# Autodesk Inventor assembly: (FINAL)rollerAssembly
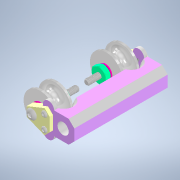
[picture p0: Inventor's stored thumbnail of the model, 180x180]
Saved by Autodesk Inventor 2022 (Build 260153000, 153)
## iProperties
Created: 2022-11-15
Part Number: (FINAL)rollerAssembly
Document SubType Name: Assembly
Designer: matia
Author: matia
## Documents named in this file (9)
- C:\Users\matia\Desktop\1QuadMod\(FINAL)rollerAssembly.iam
- C:\Users\matia\Desktop\1QuadMod\screws\92949A314_18-8 Stainless Steel Button Head Hex Drive Screw(final).ipt
- C:\Users\matia\Desktop\1QuadMod\rollers\rollerbase(v2).ipt
- C:\Users\matia\Desktop\1QuadMod\rollers\rollertriangle(v3).ipt
- C:\Users\matia\Desktop\1QuadMod\screws\92949A333_18-8 Stainless Steel Button Head Hex Drive Screw.ipt
- C:\Users\matia\Desktop\1QuadMod\rollers\wheel.ipt
- C:\Users\matia\Desktop\1QuadMod\rollers\wheelbushing.ipt
- C:\Users\matia\Desktop\1QuadMod\rollers\rollerwasher.ipt
- C:\Users\matia\Desktop\1QuadMod\screws\90480A006_Low-Strength Steel Hex Nut (.125).ipt
## Components (19 placed, 8 different names)
1. 92949A314_18-8 Stainless Steel Button Head Hex Drive Screw(final):1 — Mate:4, Mate:23
2. 92949A314_18-8 Stainless Steel Button Head Hex Drive Screw(final):2 — Mate:3, Mate:24
3. 92949A314_18-8 Stainless Steel Button Head Hex Drive Screw(final):3 — Mate:7, Mate:25
4. 92949A314_18-8 Stainless Steel Button Head Hex Drive Screw(final):4 — Mate:8, Mate:26
5. rollerbase(v2):1 — Mate:1, Mate:2, Mate:5, Mate:6
6. rollertriangle(v3):1 — Mate:1, Mate:2, Mate:3, Mate:4, Mate:9, Mate:23, Mate:24
7. rollertriangle(v3):2 — Mate:5, Mate:6, Mate:7, Mate:8, Mate:10, Mate:25, Mate:26
8. 92949A333_18-8 Stainless Steel Button Head Hex Drive Screw:1 — Mate:10, Mate:15, Mate:16, Mate:19, Mate:20, Mate:22
9. 92949A333_18-8 Stainless Steel Button Head Hex Drive Screw:2 — Mate:9, Mate:17, Mate:18, Mate:21
10. wheel:1 — Mate:11, Mate:12
11. wheel:2 — Mate:13, Mate:14
12. wheelbushing:1 — Mate:11, Mate:12, Mate:16
13. wheelbushing:2 — Mate:13, Mate:14, Mate:15
14. rollerwasher:1 — Mate:17
15. rollerwasher:2 — Mate:18
16. rollerwasher:3 — Mate:19
17. rollerwasher:4 — Mate:20
18. 90480A006_Low-Strength Steel Hex Nut (.125):1 — Mate:21
19. 90480A006_Low-Strength Steel Hex Nut (.125):2 — Mate:22
## Relationships (26: Mate 26)
- Mate:1: rollerbase(v2):1 ↔ rollertriangle(v3):1
- Mate:2: rollerbase(v2):1 ↔ rollertriangle(v3):1
- Mate:3: 92949A314_18-8 Stainless Steel Button Head Hex Drive Screw(final):2 ↔ rollertriangle(v3):1
- Mate:4: 92949A314_18-8 Stainless Steel Button Head Hex Drive Screw(final):1 ↔ rollertriangle(v3):1
- Mate:5: rollerbase(v2):1 ↔ rollertriangle(v3):2
- Mate:6: rollerbase(v2):1 ↔ rollertriangle(v3):2
- Mate:7: 92949A314_18-8 Stainless Steel Button Head Hex Drive Screw(final):3 ↔ rollertriangle(v3):2
- Mate:8: 92949A314_18-8 Stainless Steel Button Head Hex Drive Screw(final):4 ↔ rollertriangle(v3):2
- Mate:9: rollertriangle(v3):1 ↔ 92949A333_18-8 Stainless Steel Button Head Hex Drive Screw:2
- Mate:10: rollertriangle(v3):2 ↔ 92949A333_18-8 Stainless Steel Button Head Hex Drive Screw:1
- Mate:11: wheel:1 ↔ wheelbushing:1
- Mate:12: wheel:1 ↔ wheelbushing:1
- Mate:13: wheel:2 ↔ wheelbushing:2
- Mate:14: wheel:2 ↔ wheelbushing:2
- Mate:15: 92949A333_18-8 Stainless Steel Button Head Hex Drive Screw:1 ↔ wheelbushing:2
- Mate:16: 92949A333_18-8 Stainless Steel Button Head Hex Drive Screw:1 ↔ wheelbushing:1
- Mate:17: 92949A333_18-8 Stainless Steel Button Head Hex Drive Screw:2 ↔ rollerwasher:1
- Mate:18: 92949A333_18-8 Stainless Steel Button Head Hex Drive Screw:2 ↔ rollerwasher:2
- Mate:19: 92949A333_18-8 Stainless Steel Button Head Hex Drive Screw:1 ↔ rollerwasher:3
- Mate:20: 92949A333_18-8 Stainless Steel Button Head Hex Drive Screw:1 ↔ rollerwasher:4
- Mate:21: 92949A333_18-8 Stainless Steel Button Head Hex Drive Screw:2 ↔ 90480A006_Low-Strength Steel Hex Nut (.125):1
- Mate:22: 92949A333_18-8 Stainless Steel Button Head Hex Drive Screw:1 ↔ 90480A006_Low-Strength Steel Hex Nut (.125):2
- Mate:23: 92949A314_18-8 Stainless Steel Button Head Hex Drive Screw(final):1 ↔ rollertriangle(v3):1
- Mate:24: 92949A314_18-8 Stainless Steel Button Head Hex Drive Screw(final):2 ↔ rollertriangle(v3):1
- Mate:25: 92949A314_18-8 Stainless Steel Button Head Hex Drive Screw(final):3 ↔ rollertriangle(v3):2
- Mate:26: 92949A314_18-8 Stainless Steel Button Head Hex Drive Screw(final):4 ↔ rollertriangle(v3):2
